# Autodesk Inventor assembly: Overview
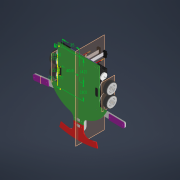
[picture p0: Inventor's stored thumbnail of the model, 180x180]
Saved by Autodesk Inventor 2022 (Build 260153000, 153)
## iProperties
Created: 2021-10-05
Part Number: Overview
Document SubType Name: Assembly
Designer: shiok
Mass: 103.359 g
Surface Area: 978.929 cm^2
Volume: 78.8399 cm^3
Density: 1.311 g/cm^3
Author: shiok
## Documents named in this file (11)
- C:\Users\shiok\Documents\GitHub\murakumo\inventor\Overview.iam
- C:\Users\shiok\Documents\GitHub\murakumo\inventor\flame.ipt
- C:\Users\shiok\Documents\GitHub\murakumo\inventor\Motor.iam
- C:\Users\shiok\Documents\GitHub\murakumo\inventor\Motor_MIR1.iam
- C:\Users\shiok\Documents\GitHub\murakumo\inventor\sensor.ipt
- C:\Users\shiok\Documents\GitHub\murakumo\inventor\SideSensor.ipt
- C:\Users\shiok\Documents\GitHub\murakumo\inventor\SideSensorCircuit.ipt
- C:\Users\shiok\Documents\GitHub\murakumo\inventor\SideSensor_MIR.ipt
- C:\Users\shiok\Documents\GitHub\murakumo\inventor\SideSensorCircuit_MIR1.ipt
- C:\Users\shiok\Documents\GitHub\murakumo\inventor\top.ipt
- C:\Users\shiok\Documents\GitHub\murakumo\inventor\jump.ipt
## Components (10 placed, 10 different names)
1. flame:1 — フラッシュ:1, フラッシュ:2, フラッシュ:3, 挿入:17, 挿入:19, メイト:10, 挿入:20, メイト:11, メイト:15, フラッシュ:7, メイト:16
2. Motor:1 [sub-assembly] — 対称度:2, メイト:10, 対称度:3
3. sensor:1 — フラッシュ:6, メイト:15, フラッシュ:7, メイト:17, メイト:18
4. Motor_MIR1:1 [sub-assembly] — 挿入:17, 挿入:18, 対称度:2, 対称度:3, メイト:12, メイト:13, メイト:14
5. SideSensor:1 — 挿入:11, 挿入:12, メイト:7, 挿入:20, メイト:11
6. SideSensorCircuit:1 — 挿入:11, 挿入:12, メイト:7
7. SideSensor_MIR:1 — 挿入:15, 挿入:16, メイト:9, 挿入:18, 挿入:19
8. SideSensorCircuit_MIR1:1 — 挿入:15, 挿入:16, メイト:9
9. top:1 — メイト:12, メイト:13, メイト:14
10. jump:1 — メイト:16, メイト:17, メイト:18
## Relationships (26: Mate 11, Insert 8, Flush 5, Symmetry 2)
- フラッシュ:1 [Flush]: flame:1
- フラッシュ:2 [Flush]: flame:1
- フラッシュ:3 [Flush]: flame:1
- フラッシュ:6 [Flush]: sensor:1
- 挿入:11 [Insert]: SideSensor:1 ↔ SideSensorCircuit:1
- 挿入:12 [Insert]: SideSensor:1 ↔ SideSensorCircuit:1
- メイト:7 [Mate]: SideSensor:1 ↔ SideSensorCircuit:1
- 挿入:15 [Insert]: SideSensor_MIR:1 ↔ SideSensorCircuit_MIR1:1
- 挿入:16 [Insert]: SideSensor_MIR:1 ↔ SideSensorCircuit_MIR1:1
- メイト:9 [Mate]: SideSensor_MIR:1 ↔ SideSensorCircuit_MIR1:1
- 挿入:17 [Insert]: flame:1 ↔ Motor_MIR1:1
- 挿入:18 [Insert]: Motor_MIR1:1 ↔ SideSensor_MIR:1
- 挿入:19 [Insert]: flame:1 ↔ SideSensor_MIR:1
- 対称度:2 [Symmetry]: Motor:1 ↔ Motor_MIR1:1
- メイト:10 [Mate]: flame:1 ↔ Motor:1
- 挿入:20 [Insert]: flame:1 ↔ SideSensor:1
- メイト:11 [Mate]: flame:1 ↔ SideSensor:1
- 対称度:3 [Symmetry]: Motor:1 ↔ Motor_MIR1:1
- メイト:12 [Mate]: Motor_MIR1:1 ↔ top:1
- メイト:13 [Mate]: Motor_MIR1:1 ↔ top:1
- メイト:14 [Mate]: Motor_MIR1:1 ↔ top:1
- メイト:15 [Mate]: flame:1 ↔ sensor:1
- フラッシュ:7 [Flush]: flame:1 ↔ sensor:1
- メイト:16 [Mate]: flame:1 ↔ jump:1
- メイト:17 [Mate]: sensor:1 ↔ jump:1
- メイト:18 [Mate]: sensor:1 ↔ jump:1
